# Autodesk Inventor assembly: Housing 4
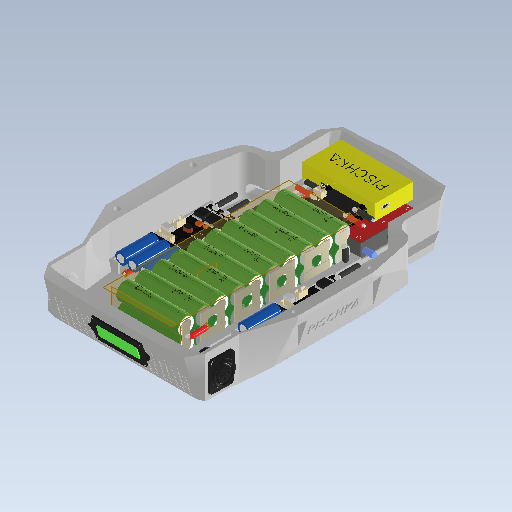
[picture p0: Inventor's stored thumbnail of the model, 512x512]
Saved by Autodesk Inventor 2020.1 (Build 241239000, 239)
## iProperties
Created: 2019-11-16
Part Number: Housing 4
Document SubType Name: Assembly
Designer: Petar
Author: Petar
## Documents named in this file (10)
- D:\OMG\E-Board\CAD\Inventor\Housing\Housing v3.iam
- D:\OMG\E-Board\CAD\Inventor\Housing\Battery Housing Box v3.ipt
- D:\OMG\E-Board\CAD\Inventor\Electrical Components\Battery Indicator.ipt
- D:\OMG\E-Board\CAD\Inventor\Electrical Components\BMS (separate port).ipt
- D:\OMG\E-Board\CAD\Inventor\Electrical Components\Battery Pack\Samsung 25R\Battery Pack - Samsung 25R - 2xRows.iam
- D:\OMG\E-Board\CAD\Inventor\Electrical Components\Power Switch - detail.ipt
- D:\OMG\E-Board\CAD\Inventor\Electrical Components\Power Button.ipt
- D:\OMG\E-Board\CAD\Inventor\Electrical Components\VESC - detail.ipt
- D:\OMG\E-Board\CAD\Inventor\Electrical Components\XLR Female Plug.ipt
- D:\OMG\E-Board\CAD\Inventor\Remote\Receiver.iam
## Components (10 placed, 9 different names)
1. Battery Housing Box v3:1 — Rigid:4, Rigid:5, Mate:2, Mate:3, Mate:4, Flush:1, Mate:5, Rigid:6, Rigid:7
2. Battery Indicator:1 — Rigid:4
3. BMS (separate port):1 — Rigid:7, Rigid:10, Rigid:11
4. Battery Pack - Samsung 25R - 2xRows:1 [sub-assembly] — Flush:1, Mate:5
5. Power Switch - detail:1 — Rigid:10
6. Power Button:1 — Rigid:6
7. VESC - detail:1
8. VESC - detail:2
9. XLR Female Plug:1 — Rigid:5
10. Receiver:1 [sub-assembly] — Rigid:11
## Relationships (11: WeldJoint 6, Mate 4, Flush 1)
- Rigid:4 [WeldJoint]: Battery Housing Box v3:1 ↔ Battery Indicator:1
- Rigid:5 [WeldJoint]: Battery Housing Box v3:1 ↔ XLR Female Plug:1
- Mate:2: Battery Housing Box v3:1
- Mate:3: Battery Housing Box v3:1
- Mate:4: Battery Housing Box v3:1
- Flush:1: Battery Housing Box v3:1 ↔ Battery Pack - Samsung 25R - 2xRows:1
- Mate:5: Battery Housing Box v3:1 ↔ Battery Pack - Samsung 25R - 2xRows:1
- Rigid:6 [WeldJoint]: Battery Housing Box v3:1 ↔ Power Button:1
- Rigid:7 [WeldJoint]: Battery Housing Box v3:1 ↔ BMS (separate port):1
- Rigid:10 [WeldJoint] (3.8 mm): BMS (separate port):1 ↔ Power Switch - detail:1
- Rigid:11 [WeldJoint]: BMS (separate port):1 ↔ Receiver:1
